# Autodesk Inventor assembly: Full_Assembly
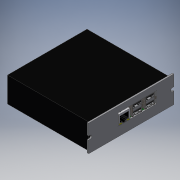
[picture p0: Inventor's stored thumbnail of the model, 180x180]
Saved by Autodesk Inventor 2016 (Build 200138000, 138)
## iProperties
Created: 2018-07-17
Part Number: Full_Assembly
Document SubType Name: Assembly
Designer: Jorian Bruslind
Author: Jorian Bruslind
## Documents named in this file (5)
- C:\Users\Jorian Bruslind\Documents\GitHub\PersonalProjects\Inventor Projects\Useful models\Full_Assembly.iam
- C:\Users\Jorian Bruslind\Documents\GitHub\PersonalProjects\Inventor Projects\Useful models\Slot.ipt
- C:\Users\Jorian Bruslind\Documents\GitHub\PersonalProjects\Inventor Projects\Useful models\Plastic_Housing.ipt
- C:\Users\Jorian Bruslind\Documents\GitHub\PersonalProjects\Inventor Projects\Useful models\Raspberry Pi 3.iam
- C:\Users\Jorian Bruslind\Documents\GitHub\PersonalProjects\Inventor Projects\Useful models\M3x6 Philips Screw.ipt
## Components (7 placed, 4 different names)
1. Slot:1 — Mate:1, Mate:2, Mate:3, Tangent:1, Tangent:4
2. Plastic_Housing:1 — Mate:1, Mate:2
3. Raspberry Pi 3:1 [sub-assembly] — Mate:3, Tangent:1, Flush:1, Tangent:2, Flush:2, Tangent:3, Tangent:4, Flush:3, Tangent:5, Flush:4, Tangent:6
4. M3x6 Philips Screw:1 — Flush:3, Tangent:5
5. M3x6 Philips Screw:2 — Flush:2, Tangent:3
6. M3x6 Philips Screw:3 — Flush:1, Tangent:2
7. M3x6 Philips Screw:4 — Flush:4, Tangent:6
## Relationships (13: Tangent 6, Flush 4, Mate 3)
- Mate:1: Slot:1 ↔ Plastic_Housing:1
- Mate:2 (2 mm): Slot:1 ↔ Plastic_Housing:1
- Mate:3: Slot:1 ↔ Raspberry Pi 3:1
- Tangent:1: Slot:1 ↔ Raspberry Pi 3:1
- Flush:1 (-1 mm): Raspberry Pi 3:1 ↔ M3x6 Philips Screw:3
- Tangent:2: Raspberry Pi 3:1 ↔ M3x6 Philips Screw:3
- Flush:2 (-1 mm): Raspberry Pi 3:1 ↔ M3x6 Philips Screw:2
- Tangent:3: Raspberry Pi 3:1 ↔ M3x6 Philips Screw:2
- Tangent:4: Slot:1 ↔ Raspberry Pi 3:1
- Flush:3 (-1 mm): Raspberry Pi 3:1 ↔ M3x6 Philips Screw:1
- Tangent:5: Raspberry Pi 3:1 ↔ M3x6 Philips Screw:1
- Flush:4 (-1 mm): Raspberry Pi 3:1 ↔ M3x6 Philips Screw:4
- Tangent:6: Raspberry Pi 3:1 ↔ M3x6 Philips Screw:4
